# Autodesk Inventor assembly: asstseal
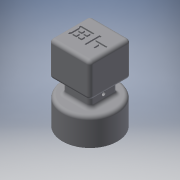
[picture p0: Inventor's stored thumbnail of the model, 180x180]
Saved by Autodesk Inventor 2019 (Build 230136000, 136)
## iProperties
Created: 2020-10-22
Part Number: asstseal
Material: 一般
Document SubType Name: Assembly
Designer: Masato
Author: Masato
## Documents named in this file (3)
- C:\Users\Masato\Documents\GitHubRepositories\asst.seal_model\asstseal.iam
- C:\Users\Masato\Documents\GitHubRepositories\asst.seal_model\asst.ipt
- C:\Users\Masato\Documents\GitHubRepositories\asst.seal_model\ueda_seal.ipt
## Components (2 placed, 2 different names)
1. asst:1 — 挿入:1, 角度:1, メイト:1
2. ueda_seal:1 — 挿入:1, 角度:1
## Relationships (3: Insert 1, Angle 1, Mate 1)
- 挿入:1 [Insert]: asst:1 ↔ ueda_seal:1
- 角度:1 [Angle] (0 deg): asst:1 ↔ ueda_seal:1
- メイト:1 [Mate]: asst:1
